# Autodesk Inventor assembly: gabinete-montagem
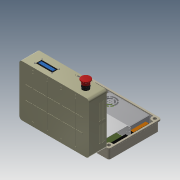
[picture p0: Inventor's stored thumbnail of the model, 180x180]
Saved by Autodesk Inventor 2017 (Build 210142000, 142)
## iProperties
Created: 2018-08-05
Part Number: gabinete-montagem
Document SubType Name: Assembly
Designer: Luiz Gustavo
Author: Luiz Gustavo
## Documents named in this file (18)
- C:\Users\Luiz Gustavo\Documents\Inventor\piano-robot\gabinete-montagem.iam
- C:\Users\Luiz Gustavo\Documents\Inventor\piano-robot\caixa-gabinete-fundo.ipt
- C:\Users\Luiz Gustavo\Documents\Inventor\piano-robot\emergency-button.ipt
- C:\Users\Luiz Gustavo\Documents\Inventor\piano-robot\lcd-16x2-display.ipt
- C:\Users\Luiz Gustavo\Documents\Inventor\piano-robot\panel-usb.ipt
- C:\Users\Luiz Gustavo\Documents\Inventor\piano-robot\power-port.ipt
- C:\Users\Luiz Gustavo\Documents\Inventor\piano-robot\caixa-gabinete-tampa.ipt
- C:\Users\Luiz Gustavo\Documents\Inventor\piano-robot\gabinete-montagem\Design Accelerator\Bolted Connection1.iam
- C:\Users\Luiz Gustavo\Documents\Inventor\piano-robot\gabinete-montagem\Design Accelerator\Bolted Connection2.iam
- C:\Users\Luiz Gustavo\Documents\Inventor\piano-robot\hdmi-cable.ipt
- C:\Users\Luiz Gustavo\Documents\Inventor\piano-robot\fonte-24v-andeli.ipt
- C:\Users\Luiz Gustavo\Documents\Inventor\piano-robot\fonte-12v-hellofish.ipt
- C:\Users\Luiz Gustavo\Documents\Inventor\piano-robot\driver WD-2404.ipt
- C:\Users\Luiz Gustavo\Documents\Inventor\piano-robot\grabcad\arduino-mega-2560-corrcted-1.snapshot.1\ArduinoMega2560 CORRECTED.ipt
- C:\Users\Luiz Gustavo\Documents\Inventor\piano-robot\grabcad\raspberry-pi-3-model-b-2.snapshot.2\Rpi3Bplus.ipt
- C:\Users\Luiz Gustavo\Documents\Inventor\piano-robot\piano-electric\piano-robot-board1.iam
- C:\Users\Luiz Gustavo\Documents\Inventor\piano-robot\piano-electric\piano-robot-board2.iam
- C:\Users\Luiz Gustavo\Documents\Inventor\piano-robot\piano-electric\piano-robot-board3.iam
## Components (21 placed, 16 different names)
1. caixa-gabinete-fundo:1 — Mate:2, Flush:2, Flush:3, Rigid:1, Rigid:2, Rigid:3, Rotational:2, Mate:3, Mate:4, Mate:5, Mate:8, Mate:9, Rotational:3, Rigid:4, Mate:23, Mate:24, Mate:25, Mate:26, Mate:27, Mate:28, Mate:29, Mate:30, Mate:31, Mate:32, Flush:6, Mate:34, Mate:35, Mate:36
2. caixa-gabinete-tampa:1 — Mate:6, Mate:7, Flush:4, Mate:12, Mate:13, Mate:14, Mate:16, Mate:17, Mate:18, Mate:19, Mate:20, Mate:21
3. emergency-button:1 — Rigid:1
4. lcd-16x2-display:1 — Mate:3, Mate:4, Mate:5
5. panel-usb:1 — Rigid:4
6. panel-usb:2 — Rigid:2
7. panel-usb:3 — Rigid:3
8. power-port:1 — Rotational:2, Mate:10, Mate:11, Mate:33
9. Bolted Connection:1 [sub-assembly] — Mate:8, Mate:9
10. Bolted Connection:2 [sub-assembly] — Mate:10, Mate:11
11. hdmi-cable:1 — Rotational:3
12. fonte-24v-andeli:1 — Mate:12, Mate:15, Mate:17
13. fonte-12v-hellofish:1 — Mate:13, Mate:14, Mate:15, Mate:16
14. driver WD-2404:1 — Mate:18, Mate:19, Mate:20, Mate:22, Flush:5
15. driver WD-2404:2 — Mate:21, Mate:22, Flush:5
16. ArduinoMega2560 CORRECTED:1 — Mate:32, Flush:6
17. Rpi3Bplus:1 — Mate:31, Mate:33
18. piano-robot-board1:1 [sub-assembly] — Mate:23, Mate:27, Mate:30
19. piano-robot-board2:1 [sub-assembly] — Mate:24, Mate:26
20. piano-robot-board3:1 [sub-assembly] — Mate:25, Mate:28, Mate:29
21. fonte-12v-hellofish:2 — Mate:34, Mate:35, Mate:36
## Relationships (46: Mate 35, Flush 5, WeldJoint 4, RevoluteJoint 2)
- Mate:2: caixa-gabinete-fundo:1
- Flush:2: caixa-gabinete-fundo:1
- Flush:3: caixa-gabinete-fundo:1
- Rigid:1 [WeldJoint]: caixa-gabinete-fundo:1 ↔ emergency-button:1
- Rigid:2 [WeldJoint]: caixa-gabinete-fundo:1 ↔ panel-usb:2
- Rigid:3 [WeldJoint]: caixa-gabinete-fundo:1 ↔ panel-usb:3
- Rotational:2 [RevoluteJoint]: caixa-gabinete-fundo:1 ↔ power-port:1
- Mate:3: caixa-gabinete-fundo:1 ↔ lcd-16x2-display:1
- Mate:4: caixa-gabinete-fundo:1 ↔ lcd-16x2-display:1
- Mate:5: caixa-gabinete-fundo:1 ↔ lcd-16x2-display:1
- Mate:6 (-115 mm): caixa-gabinete-tampa:1
- Mate:7: caixa-gabinete-tampa:1
- Flush:4 (-200 mm): caixa-gabinete-tampa:1
- Mate:8: caixa-gabinete-fundo:1 ↔ Bolted Connection:1
- Mate:9: caixa-gabinete-fundo:1 ↔ Bolted Connection:1
- Mate:10: power-port:1 ↔ Bolted Connection:2
- Mate:11: power-port:1 ↔ Bolted Connection:2
- Rotational:3 [RevoluteJoint]: caixa-gabinete-fundo:1 ↔ hdmi-cable:1
- Rigid:4 [WeldJoint]: caixa-gabinete-fundo:1 ↔ panel-usb:1
- Mate:12: caixa-gabinete-tampa:1 ↔ fonte-24v-andeli:1
- Mate:13: caixa-gabinete-tampa:1 ↔ fonte-12v-hellofish:1
- Mate:14: caixa-gabinete-tampa:1 ↔ fonte-12v-hellofish:1
- Mate:15: fonte-24v-andeli:1 ↔ fonte-12v-hellofish:1
- Mate:16: caixa-gabinete-tampa:1 ↔ fonte-12v-hellofish:1
- Mate:17: caixa-gabinete-tampa:1 ↔ fonte-24v-andeli:1
- Mate:18: caixa-gabinete-tampa:1 ↔ driver WD-2404:1
- Mate:19: caixa-gabinete-tampa:1 ↔ driver WD-2404:1
- Mate:20: caixa-gabinete-tampa:1 ↔ driver WD-2404:1
- Mate:21: caixa-gabinete-tampa:1 ↔ driver WD-2404:2
- Mate:22: driver WD-2404:1 ↔ driver WD-2404:2
- Flush:5: driver WD-2404:1 ↔ driver WD-2404:2
- Mate:23: caixa-gabinete-fundo:1 ↔ piano-robot-board1:1
- Mate:24: caixa-gabinete-fundo:1 ↔ piano-robot-board2:1
- Mate:25: caixa-gabinete-fundo:1 ↔ piano-robot-board3:1
- Mate:26: caixa-gabinete-fundo:1 ↔ piano-robot-board2:1
- Mate:27 (1.5 mm): caixa-gabinete-fundo:1 ↔ piano-robot-board1:1
- Mate:28 (1.5 mm): caixa-gabinete-fundo:1 ↔ piano-robot-board3:1
- Mate:29: caixa-gabinete-fundo:1 ↔ piano-robot-board3:1
- Mate:30: caixa-gabinete-fundo:1 ↔ piano-robot-board1:1
- Mate:31: caixa-gabinete-fundo:1 ↔ Rpi3Bplus:1
- Mate:32 (2 mm): caixa-gabinete-fundo:1 ↔ ArduinoMega2560 CORRECTED:1
- Flush:6 (20 mm): caixa-gabinete-fundo:1 ↔ ArduinoMega2560 CORRECTED:1
- Mate:33 (30 mm): power-port:1 ↔ Rpi3Bplus:1
- Mate:34: caixa-gabinete-fundo:1 ↔ fonte-12v-hellofish:2
- Mate:35: caixa-gabinete-fundo:1 ↔ fonte-12v-hellofish:2
- Mate:36: caixa-gabinete-fundo:1 ↔ fonte-12v-hellofish:2
